# Autodesk Inventor assembly: assembly
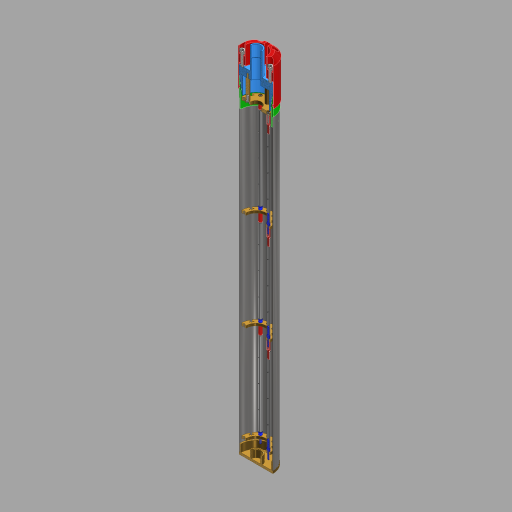
[picture p0: Inventor's stored thumbnail of the model, 512x512]
Saved by Autodesk Inventor 2024 (Build 280153020, 153B)
## iProperties
Created: 2023-09-22
Part Number: assembly
Document SubType Name: Assembly
Designer: schanen
Author: schanen
## Documents named in this file (6)
- C:\Users\schanen\Documents\Inventor\he4inserts\assembly.iam
- C:\Users\schanen\Documents\Inventor\he4inserts\Clamp.ipt
- C:\Users\schanen\Documents\Inventor\he4inserts\Screw_StainlessSteal_M4_SocketCap_20mm.ipt
- C:\Users\schanen\Documents\Inventor\he4inserts\FlangeCone.ipt
- C:\Users\schanen\Documents\Inventor\he4inserts\insertAssembly-3.iam
- C:\Users\schanen\Documents\Inventor\he4inserts\ThinBody.iam
## Components (11 placed, 5 different names)
1. Clamp:1 — Mate:1, Mate:3, Mate:4, Flush:1, Mate:5, Angle:1, Mate:17, Mate:28
2. Clamp:2 — Mate:3, Mate:4, Flush:1
3. FlangeCone:1 — Mate:5, Mate:6, Mate:7, Mate:17, Mate:27, Tangent:1, Mate:29
4. insertAssembly-3:1 [sub-assembly] — Mate:29, Mate:30
5. ThinBody:1 [sub-assembly] — Mate:27, Mate:28, Tangent:1
6. Screw_StainlessSteal_M4_SocketCap_20mm:1 — Mate:1, Mate:6
7. Screw_StainlessSteal_M4_SocketCap_20mm:2
8. Screw_StainlessSteal_M4_SocketCap_20mm:3
9. Screw_StainlessSteal_M4_SocketCap_20mm:4
10. Screw_StainlessSteal_M4_SocketCap_20mm:5
11. Screw_StainlessSteal_M4_SocketCap_20mm:6
## Component patterns: (6 elements, first: Screw_StainlessSteal_M4_SocketCap_20mm:1)
## Relationships (16: Mate 13, Flush 1, Angle 1, Tangent 1)
- Mate:1: Clamp:1 ↔ Screw_StainlessSteal_M4_SocketCap_20mm:1
- Mate:3: Clamp:1 ↔ Clamp:2
- Mate:4 (5 mm): Clamp:1 ↔ Clamp:2
- Flush:1: Clamp:1 ↔ Clamp:2
- Mate:5: Clamp:1 ↔ FlangeCone:1
- Mate:6: FlangeCone:1 ↔ Screw_StainlessSteal_M4_SocketCap_20mm:1
- Mate:7: FlangeCone:1
- Angle:1 (0 deg): Clamp:1
- Mate:17: Clamp:1 ↔ FlangeCone:1
- [Mate]: FlangeCone:1 ↔ insertAssembly-3:1
- [Mate]: FlangeCone:1 ↔ insertAssembly-3:1
- Mate:27: FlangeCone:1 ↔ ThinBody:1
- Mate:28: Clamp:1 ↔ ThinBody:1
- Tangent:1: FlangeCone:1 ↔ ThinBody:1
- Mate:29: FlangeCone:1 ↔ insertAssembly-3:1
- Mate:30: insertAssembly-3:1
